# Autodesk Inventor assembly: ASY платформа
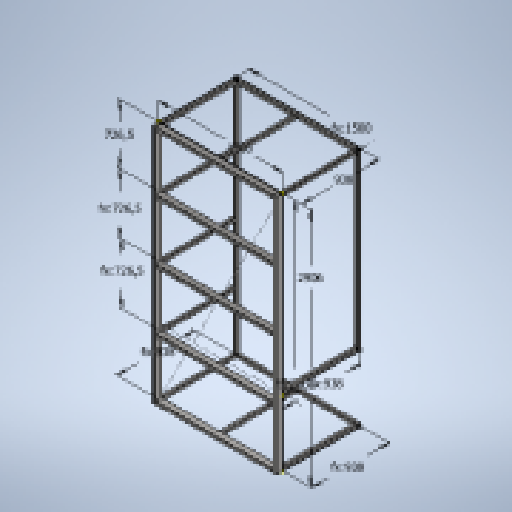
[picture p0: Inventor's stored thumbnail of the model, 512x512]
Saved by Autodesk Inventor 2025 (Build 290162010, 162A)
## iProperties
_SolveAssemblyDoc: Frame Generator Solve Assembly
_Version: 25.0.0
Created: 2025-01-19
Part Number: ASY платформа
Document SubType Name: Assembly
Designer: pokla
Author: pokla
## Documents named in this file (4)
- C:\Users\admin\YandexDisk-badmisterfox\домашниий пк\Inventor\NDM-VOS_powder_hopper\ASY платформа.iam
- C:\Users\admin\YandexDisk-badmisterfox\домашниий пк\Inventor\NDM-VOS_powder_hopper\Эскиз платформа.ipt
- C:\Users\admin\YandexDisk-badmisterfox\домашниий пк\Inventor\NDM-VOS_powder_hopper\ASY платформа\Frame\Frame 1737291159877.iam
- C:\Users\admin\YandexDisk-badmisterfox\домашниий пк\Inventor\NDM-VOS_powder_hopper\ISO 4019 - 40x40x2 - 898.ipt
## Components (9 placed, 3 different names)
1. Эскиз платформа:1
2. Frame 1737291159877:1 [sub-assembly] — Mate:1, Flush:1, Mate:2, Mate:3, Flush:2, Mate:4, Mate:5, Flush:3, Mate:6, Mate:9, Flush:5, Mate:10
3. ISO 4019 - 40x40x2 - 898:1 — Mate:1, Flush:1, Mate:2
4. ISO 4019 - 40x40x2 - 898:2 — Mate:3, Flush:2, Mate:4
5. ISO 4019 - 40x40x2 - 898:3 — Mate:5, Flush:3, Mate:6
6. ISO 4019 - 40x40x2 - 898:6
7. ISO 4019 - 40x40x2 - 898:5 — Mate:9, Flush:5, Mate:10
8. ISO 4019 - 40x40x2 - 898:7
9. ISO 4019 - 40x40x2 - 898:8
## Component patterns: (2 elements, first: ISO 4019 - 40x40x2 - 898:3), (3 elements, first: ISO 4019 - 40x40x2 - 898:5)
## Relationships (12: Mate 8, Flush 4)
- Mate:1: Frame 1737291159877:1 ↔ ISO 4019 - 40x40x2 - 898:1
- Flush:1: Frame 1737291159877:1 ↔ ISO 4019 - 40x40x2 - 898:1
- Mate:2 (690 mm): Frame 1737291159877:1 ↔ ISO 4019 - 40x40x2 - 898:1
- Mate:3: Frame 1737291159877:1 ↔ ISO 4019 - 40x40x2 - 898:2
- Flush:2: Frame 1737291159877:1 ↔ ISO 4019 - 40x40x2 - 898:2
- Mate:4 (690 mm): Frame 1737291159877:1 ↔ ISO 4019 - 40x40x2 - 898:2
- Mate:5: Frame 1737291159877:1 ↔ ISO 4019 - 40x40x2 - 898:3
- Flush:3: Frame 1737291159877:1 ↔ ISO 4019 - 40x40x2 - 898:3
- Mate:6 (666.5 mm): Frame 1737291159877:1 ↔ ISO 4019 - 40x40x2 - 898:3
- Mate:9: Frame 1737291159877:1 ↔ ISO 4019 - 40x40x2 - 898:5
- Flush:5: Frame 1737291159877:1 ↔ ISO 4019 - 40x40x2 - 898:5
- Mate:10 (666.5 mm): Frame 1737291159877:1 ↔ ISO 4019 - 40x40x2 - 898:5
